# Autodesk Inventor assembly: MotionBaseGeneric
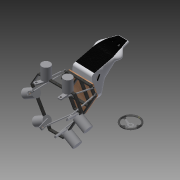
[picture p0: Inventor's stored thumbnail of the model, 180x180]
Saved by Autodesk Inventor 2015 (Build 190159000, 159)
## iProperties
Created: 2016-02-02
Part Number: MotionBaseGeneric
Document SubType Name: Assembly
Designer: tuttlem
Author: tuttlem
## Documents named in this file (11)
- C:\Users\Mac\Desktop\MotionBase\CAD\MotionBaseCAD\MotionBaseGeneric.iam
- C:\Users\Mac\Desktop\MotionBase\CAD\MotionBaseCAD\Platform.ipt
- C:\Users\Mac\Desktop\MotionBase\CAD\MotionBaseCAD\BasePlatform.ipt
- C:\Users\Mac\Desktop\MotionBase\CAD\MotionBaseCAD\Rod.ipt
- C:\Users\Mac\Desktop\MotionBase\CAD\MotionBaseCAD\Rod_MIR.ipt
- C:\Users\Mac\Desktop\MotionBase\CAD\MotionBaseCAD\arm.ipt
- C:\Users\Mac\Desktop\MotionBase\CAD\MotionBaseCAD\Motor.ipt
- C:\Users\Mac\Desktop\MotionBase\CAD\MotionBaseCAD\Bearing.ipt
- C:\Users\Mac\Desktop\MotionBase\CAD\MotionBaseCAD\PlatformTop.ipt
- C:\Users\Mac\Desktop\MotionBase\CAD\MotionBaseCAD\siege.ipt
- C:\Users\Mac\Desktop\MotionBase\CAD\MotionBaseCAD\Sparco Volante wheel.ipt
## Components (35 placed, 10 different names)
1. Platform:1 — Insert:3, Insert:5, Mate:1, Flush:7, Mate:2, Flush:8, Mate:3, Mate:4, Mate:5, Flush:9, Mate:65, Flush:20, Flush:21
2. BasePlatform:1 — Mate:6, Mate:7, Mate:8, Mate:9, Mate:10, Mate:11, Mate:12, Mate:22, Mate:23, Mate:26, Mate:27, Flush:11, Mate:41, Angle:1, Mate:44, Mate:45, Mate:46, Mate:47, Mate:48, Mate:49, Mate:52, Mate:54, Mate:55, Mate:57, Mate:58
3. PlatformTop:1 — Mate:65, Flush:20, Flush:21, Mate:66
4. siege:1 — Mate:66
5. Sparco Volante wheel:1
6. Motor:11 — Mate:9, Mate:13, Mate:37, Flush:15, Mate:59
7. Motor:10 — Mate:7, Mate:14, Mate:38, Flush:14, Angle:2, Mate:51
8. Motor:9 — Mate:12, Mate:15, Mate:35, Flush:17, Mate:56
9. Motor:8 — Mate:8, Mate:16, Mate:39, Flush:13, Angle:3, Mate:53
10. Motor:7 — Mate:11, Mate:17, Mate:36, Flush:16, Angle:4, Flush:18
11. Motor:1 — Mate:10, Mate:18, Mate:34, Flush:12, Angle:6, Flush:19
12. Rod_MIR:1 — Flush:1, Tangent:1, Mate:40
13. Rod_MIR:2 — Mate:31
14. Rod_MIR:3 — Mate:28
15. Rod_MIR:4 — Mate:29
16. Rod_MIR:5 — Mate:60
17. Rod_MIR:6 — Mate:32
18. Rod:1 — Flush:1, Tangent:1, Insert:3
19. Rod:2 — Insert:5
20. Rod:3 — Mate:1, Flush:7
21. Rod:4 — Mate:2, Flush:8
22. Rod:5 — Mate:3, Mate:4
23. Rod:6 — Mate:5, Flush:9
24. arm:1 — Mate:37, Flush:15, Mate:43
25. arm:8 — Mate:35, Flush:17, Mate:63
26. arm:9 — Mate:38, Flush:14, Mate:42
27. arm:10 — Mate:39, Flush:13, Mate:61
28. arm:11 — Mate:36, Flush:16, Mate:62
29. arm:12 — Mate:34, Flush:12, Mate:64
30. Bearing:2 — Mate:40, Mate:64
31. Bearing:3 — Mate:60, Mate:61
32. Bearing:4 — Mate:32, Mate:62
33. Bearing:5 — Mate:29, Mate:43
34. Bearing:6 — Mate:28, Mate:42
35. Bearing:1 — Mate:31, Mate:63
## Relationships (95: Mate 59, Flush 21, Angle 7, Tangent 6, Insert 2)
- Flush:1: Rod_MIR:1 ↔ Rod:1
- Tangent:1: Rod_MIR:1 ↔ Rod:1
- [Flush]: Rod_MIR:2 ↔ Rod:2
- [Tangent]: Rod_MIR:2 ↔ Rod:2
- Insert:3: Platform:1 ↔ Rod:1
- Insert:5: Platform:1 ↔ Rod:2
- [Flush]: Rod_MIR:3 ↔ Rod:3
- [Tangent]: Rod_MIR:3 ↔ Rod:3
- [Flush]: Rod_MIR:4 ↔ Rod:4
- [Tangent]: Rod_MIR:4 ↔ Rod:4
- [Flush]: Rod_MIR:5 ↔ Rod:5
- [Tangent]: Rod_MIR:5 ↔ Rod:5
- [Flush]: Rod_MIR:6 ↔ Rod:6
- [Tangent]: Rod_MIR:6 ↔ Rod:6
- Mate:1: Platform:1 ↔ Rod:3
- Flush:7: Platform:1 ↔ Rod:3
- Mate:2: Platform:1 ↔ Rod:4
- Flush:8: Platform:1 ↔ Rod:4
- Mate:3: Platform:1 ↔ Rod:5
- Mate:4: Platform:1 ↔ Rod:5
- Mate:5: Platform:1 ↔ Rod:6
- Flush:9: Platform:1 ↔ Rod:6
- Mate:6: BasePlatform:1
- Mate:7 (-254 mm): BasePlatform:1 ↔ Motor:10
- Mate:8 (-254 mm): BasePlatform:1 ↔ Motor:8
- Mate:9 (-254 mm): BasePlatform:1 ↔ Motor:11
- Mate:10 (-254 mm): BasePlatform:1 ↔ Motor:1
- Mate:11 (-254 mm): BasePlatform:1 ↔ Motor:7
- Mate:12 (-254 mm): BasePlatform:1 ↔ Motor:9
- Flush:10 (25.4 mm)
- Mate:13: Motor:11
- Mate:14: Motor:10
- Mate:15: Motor:9
- Mate:16: Motor:8
- Mate:17: Motor:7
- Mate:18: Motor:1
- Mate:22: BasePlatform:1
- Mate:23: BasePlatform:1
- Mate:26: BasePlatform:1
- Mate:27: BasePlatform:1
- Flush:11: BasePlatform:1
- Mate:28: Rod_MIR:3 ↔ Bearing:6
- Mate:29: Rod_MIR:4 ↔ Bearing:5
- Mate:31: Rod_MIR:2 ↔ Bearing:1
- Mate:32: Rod_MIR:6 ↔ Bearing:4
- Mate:34: Motor:1 ↔ arm:12
- Flush:12: Motor:1 ↔ arm:12
- Mate:35: Motor:9 ↔ arm:8
- Mate:36: Motor:7 ↔ arm:11
- Mate:37: Motor:11 ↔ arm:1
- Mate:38: Motor:10 ↔ arm:9
- Mate:39: Motor:8 ↔ arm:10
- Flush:13: Motor:8 ↔ arm:10
- Flush:14: Motor:10 ↔ arm:9
- Flush:15: Motor:11 ↔ arm:1
- Flush:16: Motor:7 ↔ arm:11
- Flush:17: Motor:9 ↔ arm:8
- Mate:40: Rod_MIR:1 ↔ Bearing:2
- Mate:41: BasePlatform:1
- Angle:1 (0 deg): BasePlatform:1
- Mate:42: arm:9 ↔ Bearing:6
- Mate:43: arm:1 ↔ Bearing:5
- Mate:44: BasePlatform:1
- Mate:45: BasePlatform:1
- Mate:46: BasePlatform:1
- Mate:47: BasePlatform:1
- Mate:48: BasePlatform:1
- Mate:49: BasePlatform:1
- Mate:50
- Angle:2 (0 deg): Motor:10
- Mate:51 (-304.8 mm): Motor:10
- Mate:52: BasePlatform:1
- Angle:3 (0 deg): Motor:8
- Mate:53: Motor:8
- Mate:54: BasePlatform:1
- Angle:4 (0 deg): Motor:7
- Mate:55: BasePlatform:1
- Angle:5 (0 deg)
- Flush:18 (-304.8 mm): Motor:7
- Mate:56: Motor:9
- Mate:57: BasePlatform:1
- Angle:6 (0 deg): Motor:1
- Mate:58: BasePlatform:1
- Angle:7 (0 deg)
- Flush:19 (-304.8 mm): Motor:1
- Mate:59: Motor:11
- Mate:60: Rod_MIR:5 ↔ Bearing:3
- Mate:61: arm:10 ↔ Bearing:3
- Mate:62: arm:11 ↔ Bearing:4
- Mate:63: arm:8 ↔ Bearing:1
- Mate:64: arm:12 ↔ Bearing:2
- Mate:65: Platform:1 ↔ PlatformTop:1
- Flush:20: Platform:1 ↔ PlatformTop:1
- Flush:21: Platform:1 ↔ PlatformTop:1
- Mate:66: PlatformTop:1 ↔ siege:1
## Named parameters: d2_d1 = 0 mm, d3_d0 = 0 mm, d18_d1 = 0 mm, d21_d0 = 0 mm, d22_d1 = 0 mm, d25_d0 = 0 mm, d26_d1 = 0 mm, d29_d0 = 0 mm, d30_d1 = 0 mm, d33_d0 = 0 mm
